# Autodesk Inventor assembly: Gearbox Mirrored
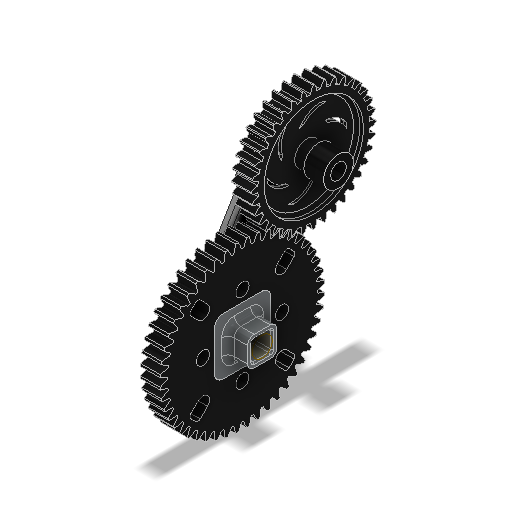
[picture p0: Inventor's stored thumbnail of the model, 512x512]
Saved by Autodesk Inventor 2025.2 (Build 292293000, 293)
## iProperties
Created: 2025-02-17
Part Number: Gearbox Mirrored
Document SubType Name: Assembly
Designer: avere
Author: avere
## Documents named in this file (12)
- C:\Users\avere\VEX-CAD\V5-CAD\Conveyer\Gearbox Mirrored.iam
- C:\Users\avere\VEX-CAD\ROBOPROS-CAD-Inventor\Motion\Gears\LS 36T Gear.ipt
- C:\Users\avere\VEX-CAD\ROBOPROS-CAD-Inventor\Motion\Spacers\Washer Steel\SWasher .375 OD x .062500.ipt
- C:\Users\avere\VEX-CAD\ROBOPROS-CAD-Inventor\Motion\Spacers\Washer Steel.ipt
- C:\Users\avere\VEX-CAD\ROBOPROS-CAD-Inventor\Motion\Spacers\Spacer Nylon .375 OD.ipt
- C:\Users\avere\VEX-CAD\ROBOPROS-CAD-Inventor\Modified Parts\Half Cut HS 48T Gear, No Insert.ipt
- C:\Users\avere\VEX-CAD\ROBOPROS-CAD-Inventor\Motion\Spacers\Spacer Nylon .375 OD\NSpacer .375 OD x .250.ipt
- C:\Users\avere\VEX-CAD\ROBOPROS-CAD-Inventor\Motion\Insert Circle.ipt
- C:\Users\avere\VEX-CAD\V5-CAD\Conveyer\Custom Parts\Gearbox Mirrored.ipt
- C:\Users\avere\VEX-CAD\ROBOPROS-CAD-Inventor\Structure\Hardware\Nut Alu.ipt
- C:\Users\avere\VEX-CAD\ROBOPROS-CAD-Inventor\Structure\Hardware\Screw Steel - Star\SScrew Star Smooth .250.ipt
- C:\Users\avere\VEX-CAD\ROBOPROS-CAD-Inventor\Structure\Hardware\Screw Steel - Star.ipt
## Components (12 placed, 8 different names)
1. LS 36T Gear:1 — Insert:23, Insert:24
2. Half Cut HS 48T Gear, No Insert:1 — Mate:5, Insert:25
3. NSpacer .375 OD x .250:5 — Insert:23
4. Insert Circle:1 — Mate:3, Mate:4, Insert:24
5. Insert Circle:2 — Mate:1, Mate:2, Mate:5
6. Gearbox Mirrored:1 — Mate:1, Mate:2, Mate:3, Mate:4, Insert:26, Mate:6, Insert:27, Insert:29
7. SWasher .375 OD x .062500:6 — Insert:25
8. Gearbox Mirrored:2 — Insert:26, Mate:6, Insert:28, Insert:30
9. Nut Alu:1 — Insert:28
10. SScrew Star Smooth .250:1 — Insert:27
11. Nut Alu:2 — Insert:30
12. SScrew Star Smooth .250:2 — Insert:29
## Relationships (14: Insert 8, Mate 6)
- Insert:23: LS 36T Gear:1 ↔ NSpacer .375 OD x .250:5
- Mate:1: Insert Circle:2 ↔ Gearbox Mirrored:1
- Mate:2: Insert Circle:2 ↔ Gearbox Mirrored:1
- Mate:3: Insert Circle:1 ↔ Gearbox Mirrored:1
- Mate:4: Insert Circle:1 ↔ Gearbox Mirrored:1
- Insert:24: LS 36T Gear:1 ↔ Insert Circle:1
- Mate:5: Half Cut HS 48T Gear, No Insert:1 ↔ Insert Circle:2
- Insert:25: Half Cut HS 48T Gear, No Insert:1 ↔ SWasher .375 OD x .062500:6
- Insert:26: Gearbox Mirrored:1 ↔ Gearbox Mirrored:2
- Mate:6: Gearbox Mirrored:1 ↔ Gearbox Mirrored:2
- Insert:27: Gearbox Mirrored:1 ↔ SScrew Star Smooth .250:1
- Insert:28: Gearbox Mirrored:2 ↔ Nut Alu:1
- Insert:29: Gearbox Mirrored:1 ↔ SScrew Star Smooth .250:2
- Insert:30: Gearbox Mirrored:2 ↔ Nut Alu:2
